# Autodesk Inventor assembly: Пандус
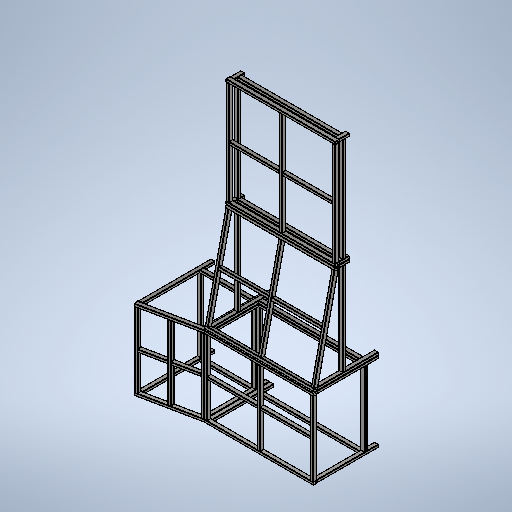
[picture p0: Inventor's stored thumbnail of the model, 512x512]
Saved by Autodesk Inventor 2025 (Build 290162010, 162A)
## iProperties
Created: 2024-09-18
Part Number: Пандус
Document SubType Name: Assembly
Designer: pokla
Author: pokla
## Documents named in this file (5)
- C:\Users\admin\YandexDisk-badmisterfox\домашниий пк\Inventor\BSH_Beshkino_bio_tank\Пандус.iam
- C:\Users\admin\YandexDisk-badmisterfox\домашниий пк\Inventor\BSH_Beshkino_bio_tank\Assembly2.iam
- C:\Users\admin\YandexDisk-badmisterfox\домашниий пк\Inventor\BSH_Beshkino_bio_tank\Assembly4.iam
- C:\Users\admin\YandexDisk-badmisterfox\домашниий пк\Inventor\BSH_Beshkino_bio_tank\Assembly6.iam
- C:\Users\admin\YandexDisk-badmisterfox\домашниий пк\Inventor\BSH_Beshkino_bio_tank\Assembly8.iam
## Components (4 placed, 4 different names)
1. Assembly2:1 [sub-assembly]
2. Assembly4:1 [sub-assembly]
3. Assembly6:1 [sub-assembly]
4. Assembly8:1 [sub-assembly]
## Relationships (3: WeldJoint 3)
- [WeldJoint]: Assembly2:1 ↔ Assembly4:1
- [WeldJoint]: Assembly6:1 ↔ Assembly8:1
- [WeldJoint]: Assembly4:1 ↔ Assembly8:1
